# Autodesk Inventor assembly: MAT BICH
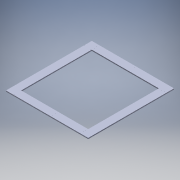
[picture p0: Inventor's stored thumbnail of the model, 180x180]
Saved by Autodesk Inventor 2017 (Build 210142000, 142)
## iProperties
Created: 2013-02-22
Part Number: MAT BICH
Document SubType Name: Assembly
Designer: XuZhiqing
Sending System: SolidWorks 2013
Last Author: Usr01
Last Saved: 2013-02-22
Author: XuZhiqing
## Documents named in this file (3)
- C:\Users\XuZhiqing\Desktop\Project01-CFD_the_sys\CAD-IPT\compressor\MAT BICH.iam
- C:\Users\XuZhiqing\Desktop\Project01-CFD_the_sys\CAD-IPT\compressor\LA.ipt
- C:\Users\XuZhiqing\Desktop\Project01-CFD_the_sys\CAD-IPT\compressor\LA_2.ipt
## Components (6 placed, 1 different names)
1. LA:1 — Flush:1, Flush:2, Flush:4, Flush:5, Flush:15
2. LA:2 — Flush:10, Flush:11, Flush:12, Flush:13, Flush:14
3. LA:3 — Flush:3, Flush:6, Flush:7, Mate:1, Flush:8, Flush:9
4. LA:4 — Flush:4, Flush:5, Flush:6, Flush:7, Mate:1, Flush:15
5. LA:4 — Flush:1, Flush:2, Flush:10, Flush:11
6. LA:5 — Flush:3, Flush:8, Flush:9, Flush:12, Flush:13, Flush:14
## Relationships (16: Flush 15, Mate 1)
- Flush:1: LA:1 ↔ LA:4
- Flush:2: LA:1 ↔ LA:4
- Flush:3: LA:3 ↔ LA:5
- Flush:4: LA:1 ↔ LA:4
- Flush:5: LA:1 ↔ LA:4
- Flush:6: LA:3 ↔ LA:4
- Flush:7: LA:3 ↔ LA:4
- Mate:1: LA:3 ↔ LA:4
- Flush:8: LA:3 ↔ LA:5
- Flush:9: LA:3 ↔ LA:5
- Flush:10: LA:2 ↔ LA:4
- Flush:11: LA:2 ↔ LA:4
- Flush:12: LA:2 ↔ LA:5
- Flush:13: LA:2 ↔ LA:5
- Flush:14: LA:2 ↔ LA:5
- Flush:15: LA:1 ↔ LA:4
